# Autodesk Inventor assembly: watercooler_fixed
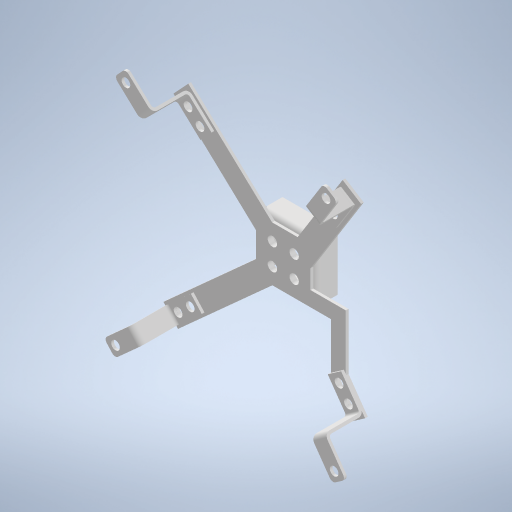
[picture p0: Inventor's stored thumbnail of the model, 512x512]
Saved by Autodesk Inventor 2023 (Build 270158000, 158)
## iProperties
Created: 2023-06-13
Part Number: watercooler_fixed
Document SubType Name: Assembly
Designer: 310611102
Author: 310611102
## Documents named in this file (4)
- C:\Users\310611102\Documents\Inventor\SSR\avionics_2023ver\electronics\watercooler_fixed.iam
- C:\Users\310611102\Documents\Inventor\SSR\avionics_2023ver\electronics\watercooler_fixed1.ipt
- C:\Users\310611102\Documents\Inventor\SSR\avionics_2023ver\electronics\watercooler_fixed2.ipt
- C:\Users\310611102\Documents\Inventor\SSR\avionics_2023ver\electronics\connector_cooler.ipt
## Components (6 placed, 3 different names)
1. watercooler_fixed1:1 — Insert:1, Insert:2
2. watercooler_fixed2:1 — Insert:1, Insert:2, Insert:3, Insert:4, Insert:5, Angle:1, Angle:3, Angle:4, Angle:5
3. connector_cooler:1 — Insert:3, Angle:5
4. connector_cooler:2 — Angle:4
5. connector_cooler:3 — Insert:4, Angle:1
6. connector_cooler:4 — Insert:5, Angle:3
## Relationships (9: Insert 5, Angle 4)
- Insert:1: watercooler_fixed1:1 ↔ watercooler_fixed2:1
- Insert:2: watercooler_fixed1:1 ↔ watercooler_fixed2:1
- Insert:3: watercooler_fixed2:1 ↔ connector_cooler:1
- Insert:4: watercooler_fixed2:1 ↔ connector_cooler:3
- Insert:5: watercooler_fixed2:1 ↔ connector_cooler:4
- Angle:1 (0 deg): watercooler_fixed2:1 ↔ connector_cooler:3
- Angle:3 (0 deg): watercooler_fixed2:1 ↔ connector_cooler:4
- Angle:4 (0 deg): watercooler_fixed2:1 ↔ connector_cooler:2
- Angle:5 (0 deg): watercooler_fixed2:1 ↔ connector_cooler:1
